# Autodesk Inventor assembly: Serial_ensamble
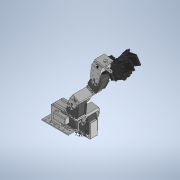
[picture p0: Inventor's stored thumbnail of the model, 180x180]
Saved by Autodesk Inventor 2021.4 (Build 254397000, 397)
## iProperties
Created: 2022-01-25
Part Number: Serial_ensamble
Document SubType Name: Assembly
Designer: epm01
Author: epm01
## Documents named in this file (8)
- D:\Archivos\2020-2\Papime\Banco_serial\Serial_ensamble.iam
- D:\Archivos\2020-2\Papime\Banco_serial\Base_serial.ipt
- D:\Archivos\2020-2\Papime\Banco_serial\AX-12A.iam
- D:\Archivos\2020-2\Papime\Banco_serial\BPF-BU.ipt
- D:\Archivos\2020-2\Papime\Banco_serial\Interfas_2.iam
- D:\Archivos\2020-2\Papime\Banco_serial\Interfas_3.iam
- D:\Archivos\2020-2\Papime\Banco_serial\Interfas_4.iam
- D:\Archivos\2020-2\Papime\Banco_serial\Gripper_re.iam
## Components (11 placed, 7 different names)
1. Base_serial:1 — Coincidencia:1, Coincidencia:2, Coincidencia:3
2. AX-12A:1 [sub-assembly] — Coincidencia:1, Coincidencia:2, Coincidencia:3, Insertar:1
3. BPF-BU:1 — Insertar:2
4. Interfas_2:1 [sub-assembly] — Insertar:1, Insertar:2, Coincidencia:4, Coincidencia:5, Coincidencia:6
5. AX-12A:2 [sub-assembly] — Coincidencia:4, Coincidencia:5, Insertar:3, Coincidencia:6
6. Interfas_3:1 [sub-assembly] — Insertar:3, Coincidencia:7, Coincidencia:8, Coincidencia:9
7. AX-12A:3 [sub-assembly] — Coincidencia:7, Coincidencia:8, Coincidencia:9, Insertar:4
8. Interfas_3:2 [sub-assembly] — Insertar:4, Coincidencia:11, Insertar:5
9. AX-12A:4 [sub-assembly] — Coincidencia:11, Insertar:5, Insertar:6
10. Interfas_4:1 [sub-assembly] — Insertar:6, Nivelación:1, Nivelación:2, Nivelación:3
11. Gripper_re:1 [sub-assembly] — Nivelación:1, Nivelación:2, Nivelación:3
## Relationships (19: Mate 10, Insert 6, Flush 3)
- Coincidencia:1 [Mate]: Base_serial:1 ↔ AX-12A:1
- Coincidencia:2 [Mate]: Base_serial:1 ↔ AX-12A:1
- Coincidencia:3 [Mate]: Base_serial:1 ↔ AX-12A:1
- Insertar:1: AX-12A:1 ↔ Interfas_2:1
- Insertar:2: BPF-BU:1 ↔ Interfas_2:1
- Coincidencia:4 [Mate]: Interfas_2:1 ↔ AX-12A:2
- Coincidencia:5 [Mate]: Interfas_2:1 ↔ AX-12A:2
- Insertar:3: AX-12A:2 ↔ Interfas_3:1
- Coincidencia:6 [Mate]: Interfas_2:1 ↔ AX-12A:2
- Coincidencia:7 [Mate]: Interfas_3:1 ↔ AX-12A:3
- Coincidencia:8 [Mate]: Interfas_3:1 ↔ AX-12A:3
- Coincidencia:9 [Mate]: Interfas_3:1 ↔ AX-12A:3
- Insertar:4: AX-12A:3 ↔ Interfas_3:2
- Coincidencia:11 [Mate]: Interfas_3:2 ↔ AX-12A:4
- Insertar:5: Interfas_3:2 ↔ AX-12A:4
- Insertar:6: AX-12A:4 ↔ Interfas_4:1
- Nivelación:1 [Flush]: Interfas_4:1 ↔ Gripper_re:1
- Nivelación:2 [Flush]: Interfas_4:1 ↔ Gripper_re:1
- Nivelación:3 [Flush]: Interfas_4:1 ↔ Gripper_re:1
